# Autodesk Inventor assembly: Staffa Modulo Fotovoltaico
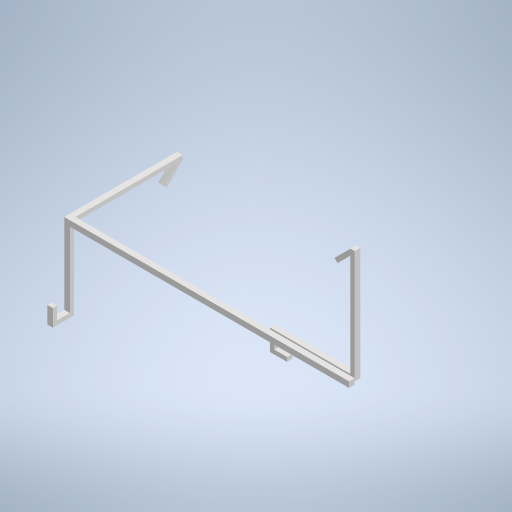
[picture p0: Inventor's stored thumbnail of the model, 512x512]
Saved by Autodesk Inventor 2024 (Build 280153000, 153)
## iProperties
Created: 2023-12-30
Part Number: Staffa Modulo Fotovoltaico
Document SubType Name: Weldment
Designer: Leonardo
Weld Material: Welded Aluminum-6061
Author: Leonardo
## Documents named in this file (4)
- C:\Users\Leonardo\Documents\Monopattino\Staffa Modulo Fotovoltaico.iam
- C:\Users\Leonardo\Documents\Monopattino\Staffa.ipt
- C:\Users\Leonardo\Documents\Monopattino\Lama.ipt
- C:\Users\Leonardo\Documents\Monopattino\Staffa_CPY.ipt
## Components (3 placed, 3 different names)
1. Staffa:1 — Rigido:1, Rigido:2
2. Lama:1 — Rigido:1, Rigido:2, Rigido:3
3. Staffa_CPY:1 — Rigido:3
## Relationships (3: WeldJoint 3)
- Rigido:1 [WeldJoint]: Staffa:1 ↔ Lama:1
- Rigido:2 [WeldJoint]: Staffa:1 ↔ Lama:1
- Rigido:3 [WeldJoint]: Lama:1 ↔ Staffa_CPY:1
